# Autodesk Inventor assembly: Assemble
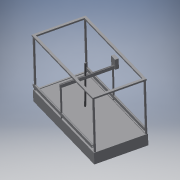
[picture p0: Inventor's stored thumbnail of the model, 180x180]
Saved by Autodesk Inventor 2017 (Build 210142000, 142)
## iProperties
Created: 2016-11-26
Part Number: Assemble
Document SubType Name: Assembly
Designer: umr
Author: umr
## Documents named in this file (8)
- D:\SeniorProject\Models\Assemble.iam
- D:\SeniorProject\Models\Base.ipt
- D:\SeniorProject\Models\wheelRoad.ipt
- D:\SeniorProject\Models\GantryRod.ipt
- D:\SeniorProject\Models\wheelRoadGantry.ipt
- D:\SeniorProject\Models\ScrewDriver.ipt
- D:\SeniorProject\Models\LedSystem.ipt
- D:\SeniorProject\Models\ElectronicCase.ipt
## Components (10 placed, 7 different names)
1. Base:1 — Mate:1, Flush:1, Flush:2, Flush:3, Flush:4, Flush:5, Mate:2, Flush:6, Flush:7, Mate:4, Mate:5, Tangent:4
2. wheelRoad:1 — Flush:2, Flush:3, Tangent:3
3. wheelRoad:2 — Flush:4, Flush:5, Tangent:5
4. GantryRod:2 — Tangent:2, Flush:9, Mate:5, Tangent:5, Tangent:6
5. GantryRod:3 — Flush:8, Tangent:1, Tangent:3, Mate:4, Tangent:7
6. wheelRoadGantry:1 — Mate:3, Flush:8, Tangent:1, Tangent:2, Flush:9, Tangent:6, Tangent:7, Flush:10, Tangent:8
7. ScrewDriver:1 — Tangent:8
8. LedSystem:1 — Mate:1, Flush:1, Tangent:4
9. ElectronicCase:1 — Mate:2, Flush:6, Flush:7
10. ElectronicCase:2 — Mate:3, Flush:10
## Relationships (23: Flush 10, Tangent 8, Mate 5)
- Mate:1: Base:1 ↔ LedSystem:1
- Flush:1: Base:1 ↔ LedSystem:1
- Flush:2: Base:1 ↔ wheelRoad:1
- Flush:3: Base:1 ↔ wheelRoad:1
- Flush:4: Base:1 ↔ wheelRoad:2
- Flush:5: Base:1 ↔ wheelRoad:2
- Mate:2: Base:1 ↔ ElectronicCase:1
- Flush:6: Base:1 ↔ ElectronicCase:1
- Flush:7 (500 mm): Base:1 ↔ ElectronicCase:1
- Mate:3: wheelRoadGantry:1 ↔ ElectronicCase:2
- Flush:8: GantryRod:3 ↔ wheelRoadGantry:1
- Tangent:1: GantryRod:3 ↔ wheelRoadGantry:1
- Tangent:2: GantryRod:2 ↔ wheelRoadGantry:1
- Flush:9: GantryRod:2 ↔ wheelRoadGantry:1
- Tangent:3: wheelRoad:1 ↔ GantryRod:3
- Mate:4: Base:1 ↔ GantryRod:3
- Mate:5: Base:1 ↔ GantryRod:2
- Tangent:4: Base:1 ↔ LedSystem:1
- Tangent:5: wheelRoad:2 ↔ GantryRod:2
- Tangent:6: GantryRod:2 ↔ wheelRoadGantry:1
- Tangent:7: GantryRod:3 ↔ wheelRoadGantry:1
- Flush:10 (-50 mm): wheelRoadGantry:1 ↔ ElectronicCase:2
- Tangent:8: wheelRoadGantry:1 ↔ ScrewDriver:1
